(part 1 of 2)
# Autodesk Inventor assembly: 110033226_iam_11_農田
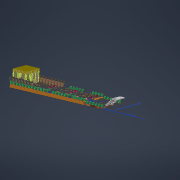
[picture p0: Inventor's stored thumbnail of the model, 180x180]
Saved by Autodesk Inventor 2022 (Build 260153000, 153)
## iProperties
Created: 2022-06-28
Part Number: 110033226_iam_11_農田
Document SubType Name: Assembly
Designer: User
Author: User
## Documents named in this file (13)
- D:\D-disk\pomelo\大一\下學期\機械設計製圖\1100332260_LEGOproj_沒有公主城堡\110033226_iam_11_農田.iam
- D:\D-disk\pomelo\大一\下學期\機械設計製圖\1100332260_LEGOproj_沒有公主城堡\110033226_ipt_44_農田基地.ipt
- D:\D-disk\pomelo\大一\下學期\機械設計製圖\1100332260_LEGOproj_沒有公主城堡\110033226_ipt_21_柵欄.ipt
- D:\D-disk\pomelo\大一\下學期\機械設計製圖\1100332260_LEGOproj_沒有公主城堡\110033226_ipt_04_小河.ipt
- D:\D-disk\pomelo\大一\下學期\機械設計製圖\1100332260_LEGOproj_沒有公主城堡\110033226_ipt_07_磚塊樺木(2x1).ipt
- D:\D-disk\pomelo\大一\下學期\機械設計製圖\1100332260_LEGOproj_沒有公主城堡\110033226_ipt_13_草地二.ipt
- D:\D-disk\pomelo\大一\下學期\機械設計製圖\1100332260_LEGOproj_沒有公主城堡\110033226_ipt_06_磚塊樺木(1x1).ipt
- D:\D-disk\pomelo\大一\下學期\機械設計製圖\1100332260_LEGOproj_沒有公主城堡\110033226_ipt_12_平滑面(2x1).ipt
- D:\D-disk\pomelo\大一\下學期\機械設計製圖\1100332260_LEGOproj_沒有公主城堡\110033226_ipt_08_平滑面(3x1).ipt
- D:\D-disk\pomelo\大一\下學期\機械設計製圖\1100332260_LEGOproj_沒有公主城堡\110033226_ipt_38_小樹木.ipt
- D:\D-disk\pomelo\大一\下學期\機械設計製圖\1100332260_LEGOproj_沒有公主城堡\110033226_ipt_45_小農田基地.ipt
- D:\D-disk\pomelo\大一\下學期\機械設計製圖\1100332260_LEGOproj_沒有公主城堡\110033226_ipt_11_樓梯支架.ipt
- D:\D-disk\pomelo\大一\下學期\機械設計製圖\1100332260_LEGOproj_沒有公主城堡\110033226_ipt_37_小河方塊.ipt
## Components (828 placed, 12 different names)
1. 110033226_ipt_38_小樹木:1 — 貼合:91, 貼合:92, 貼合:93, 貼合:96
2. 110033226_ipt_45_小農田基地:1 — 貼合:99, 貼合:100, 貼合:101, 貼合:102, 貼合:103, 貼合:104, 貼合:105, 貼合:106, 貼合:107, 貼合:108, 貼合:109, 貼合:110, 貼合:111, 貼合:112, 貼合:113, 貼合:130, 貼合:131, 貼合:135, 貼合:136, 貼合:137, 貼合:138, 貼合:139, 貼合:140, 貼合:141, 貼合:142, 貼合:146
3. 110033226_ipt_21_柵欄:50 — 貼合:108, 貼合:109, 貼合:110
4. 110033226_ipt_44_農田基地:1 — 貼合:1, 貼合:2, 貼合:3, 貼合:99, 貼合:100, 貼合:101
5. 110033226_ipt_44_農田基地:2
6. 110033226_ipt_44_農田基地:3 — 貼合:4, 貼合:5, 貼合:6, 貼合:7, 貼合:8, 貼合:9, 貼合:10, 貼合:11, 貼合:12, 貼合:13, 貼合:14, 貼合:15, 貼合:16, 貼合:17, 貼合:18, 貼合:19, 貼合:21, 貼合:22, 貼合:24, 貼合:25, 貼合:26, 貼合:27, 貼合:28, 貼合:29, 貼合:30, 貼合:31, 貼合:32, 貼合:33, 貼合:34, 貼合:35, 貼合:36, 貼合:37, 貼合:38, 貼合:39, 貼合:40, 貼合:41, 貼合:42, 貼合:43, 貼合:44, 貼合:45, 貼合:46, 貼合:47, 貼合:48, 貼合:49, 貼合:50, 貼合:88, 貼合:89, 貼合:90, 貼合:91, 貼合:92, 貼合:93, 貼合:94, 貼合:95, 貼合:97, 貼合:98
7. 110033226_ipt_04_小河:1 — 貼合:5, 貼合:6, 貼合:7
8. 110033226_ipt_04_小河:4
9. 110033226_ipt_04_小河:5
10. 110033226_ipt_04_小河:6
11. 110033226_ipt_04_小河:7
12. 110033226_ipt_04_小河:8
13. 110033226_ipt_04_小河:9
14. 110033226_ipt_04_小河:10
15. 110033226_ipt_04_小河:11
16. 110033226_ipt_04_小河:12
17. 110033226_ipt_04_小河:13
18. 110033226_ipt_04_小河:14
19. 110033226_ipt_04_小河:3 — 貼合:8, 貼合:9, 貼合:20
20. 110033226_ipt_04_小河:15 — 貼合:23
21. 110033226_ipt_04_小河:16
22. 110033226_ipt_04_小河:17
23. 110033226_ipt_04_小河:18
24. 110033226_ipt_04_小河:19
25. 110033226_ipt_04_小河:20
26. 110033226_ipt_04_小河:21
27. 110033226_ipt_04_小河:22
28. 110033226_ipt_04_小河:23
29. 110033226_ipt_04_小河:24
30. 110033226_ipt_04_小河:25
31. 110033226_ipt_21_柵欄:15 — 貼合:21, 貼合:22, 貼合:23
32. 110033226_ipt_21_柵欄:27
33. 110033226_ipt_07_磚塊樺木(2x1):1 — 貼合:24, 貼合:25, 貼合:26
34. 110033226_ipt_07_磚塊樺木(2x1):6
35. 110033226_ipt_07_磚塊樺木(2x1):7
36. 110033226_ipt_07_磚塊樺木(2x1):8
37. 110033226_ipt_07_磚塊樺木(2x1):9
38. 110033226_ipt_07_磚塊樺木(2x1):10
39. 110033226_ipt_07_磚塊樺木(2x1):11
40. 110033226_ipt_07_磚塊樺木(2x1):12
41. 110033226_ipt_07_磚塊樺木(2x1):13
42. 110033226_ipt_07_磚塊樺木(2x1):3 — 貼合:27, 貼合:28, 貼合:29
43. 110033226_ipt_07_磚塊樺木(2x1):14
44. 110033226_ipt_07_磚塊樺木(2x1):15
45. 110033226_ipt_07_磚塊樺木(2x1):16
46. 110033226_ipt_07_磚塊樺木(2x1):17
47. 110033226_ipt_07_磚塊樺木(2x1):18
48. 110033226_ipt_07_磚塊樺木(2x1):19
49. 110033226_ipt_07_磚塊樺木(2x1):20
50. 110033226_ipt_07_磚塊樺木(2x1):21
51. 110033226_ipt_07_磚塊樺木(2x1):5 — 貼合:30, 貼合:31, 貼合:32
52. 110033226_ipt_07_磚塊樺木(2x1):22
53. 110033226_ipt_07_磚塊樺木(2x1):23
54. 110033226_ipt_07_磚塊樺木(2x1):24
55. 110033226_ipt_07_磚塊樺木(2x1):25
56. 110033226_ipt_07_磚塊樺木(2x1):26
57. 110033226_ipt_07_磚塊樺木(2x1):27
58. 110033226_ipt_07_磚塊樺木(2x1):28
59. 110033226_ipt_07_磚塊樺木(2x1):2 — 貼合:33, 貼合:34, 貼合:35
60. 110033226_ipt_07_磚塊樺木(2x1):29
61. 110033226_ipt_07_磚塊樺木(2x1):30
62. 110033226_ipt_07_磚塊樺木(2x1):31
63. 110033226_ipt_07_磚塊樺木(2x1):32
64. 110033226_ipt_07_磚塊樺木(2x1):33
65. 110033226_ipt_07_磚塊樺木(2x1):4 — 貼合:36, 貼合:37, 貼合:38
66. 110033226_ipt_07_磚塊樺木(2x1):34
67. 110033226_ipt_07_磚塊樺木(2x1):35
68. 110033226_ipt_13_草地二:1 — 貼合:39, 貼合:40, 貼合:41
69. 110033226_ipt_13_草地二:2
70. 110033226_ipt_13_草地二:3
71. 110033226_ipt_13_草地二:4
72. 110033226_ipt_13_草地二:5
73. 110033226_ipt_13_草地二:6
74. 110033226_ipt_13_草地二:7
75. 110033226_ipt_13_草地二:8
76. 110033226_ipt_13_草地二:9
77. 110033226_ipt_13_草地二:10
78. 110033226_ipt_13_草地二:12 — 貼合:42, 貼合:43, 貼合:44
79. 110033226_ipt_13_草地二:13
80. 110033226_ipt_13_草地二:14
81. 110033226_ipt_13_草地二:15
82. 110033226_ipt_13_草地二:16
83. 110033226_ipt_13_草地二:17
84. 110033226_ipt_13_草地二:18
85. 110033226_ipt_13_草地二:19
86. 110033226_ipt_13_草地二:20
87. 110033226_ipt_13_草地二:21
88. 110033226_ipt_13_草地二:11 — 貼合:45, 貼合:46, 貼合:47
89. 110033226_ipt_13_草地二:22
90. 110033226_ipt_13_草地二:23
91. 110033226_ipt_13_草地二:24
92. 110033226_ipt_13_草地二:25
93. 110033226_ipt_13_草地二:26
94. 110033226_ipt_07_磚塊樺木(2x1):38 — 貼合:48, 貼合:49, 貼合:51, 貼合:52, 貼合:77
95. 110033226_ipt_06_磚塊樺木(1x1):3 — 貼合:50, 貼合:51, 貼合:52
96. 110033226_ipt_07_磚塊樺木(2x1):39
97. 110033226_ipt_06_磚塊樺木(1x1):4
98. 110033226_ipt_07_磚塊樺木(2x1):40
99. 110033226_ipt_06_磚塊樺木(1x1):5
100. 110033226_ipt_07_磚塊樺木(2x1):41
101. 110033226_ipt_06_磚塊樺木(1x1):6
102. 110033226_ipt_07_磚塊樺木(2x1):42
103. 110033226_ipt_06_磚塊樺木(1x1):7
104. 110033226_ipt_07_磚塊樺木(2x1):43
105. 110033226_ipt_06_磚塊樺木(1x1):8 — 貼合:62, 貼合:63, 貼合:64
106. 110033226_ipt_07_磚塊樺木(2x1):44
107. 110033226_ipt_06_磚塊樺木(1x1):9 — 貼合:60
108. 110033226_ipt_07_磚塊樺木(2x1):45
109. 110033226_ipt_06_磚塊樺木(1x1):10 — 貼合:59, 貼合:61
110. 110033226_ipt_07_磚塊樺木(2x1):46 — 貼合:55, 貼合:56
111. 110033226_ipt_06_磚塊樺木(1x1):11 — 貼合:53, 貼合:54
112. 110033226_ipt_07_磚塊樺木(2x1):47 — 貼合:78, 貼合:80, 貼合:81
113. 110033226_ipt_06_磚塊樺木(1x1):12
114. 110033226_ipt_07_磚塊樺木(2x1):48
115. 110033226_ipt_06_磚塊樺木(1x1):13
116. 110033226_ipt_07_磚塊樺木(2x1):49
117. 110033226_ipt_06_磚塊樺木(1x1):14
118. 110033226_ipt_07_磚塊樺木(2x1):50
119. 110033226_ipt_06_磚塊樺木(1x1):15
120. 110033226_ipt_07_磚塊樺木(2x1):51
121. 110033226_ipt_06_磚塊樺木(1x1):16
122. 110033226_ipt_07_磚塊樺木(2x1):52
123. 110033226_ipt_06_磚塊樺木(1x1):17
124. 110033226_ipt_07_磚塊樺木(2x1):53 — 貼合:86
125. 110033226_ipt_06_磚塊樺木(1x1):18
126. 110033226_ipt_07_磚塊樺木(2x1):54 — 貼合:85, 貼合:87
127. 110033226_ipt_06_磚塊樺木(1x1):19
128. 110033226_ipt_07_磚塊樺木(2x1):55
129. 110033226_ipt_06_磚塊樺木(1x1):20
130. 110033226_ipt_07_磚塊樺木(2x1):56 — 貼合:69, 貼合:71, 貼合:72, 貼合:73
131. 110033226_ipt_06_磚塊樺木(1x1):21
132. 110033226_ipt_07_磚塊樺木(2x1):57
133. 110033226_ipt_06_磚塊樺木(1x1):22
134. 110033226_ipt_07_磚塊樺木(2x1):58
135. 110033226_ipt_06_磚塊樺木(1x1):23
136. 110033226_ipt_07_磚塊樺木(2x1):59
137. 110033226_ipt_06_磚塊樺木(1x1):24
138. 110033226_ipt_07_磚塊樺木(2x1):60
139. 110033226_ipt_06_磚塊樺木(1x1):25
140. 110033226_ipt_07_磚塊樺木(2x1):61
141. 110033226_ipt_06_磚塊樺木(1x1):26 — 貼合:82
142. 110033226_ipt_07_磚塊樺木(2x1):62
143. 110033226_ipt_06_磚塊樺木(1x1):27
144. 110033226_ipt_07_磚塊樺木(2x1):63
145. 110033226_ipt_06_磚塊樺木(1x1):28
146. 110033226_ipt_07_磚塊樺木(2x1):64
147. 110033226_ipt_06_磚塊樺木(1x1):29
148. 110033226_ipt_07_磚塊樺木(2x1):65 — 貼合:68, 貼合:70
149. 110033226_ipt_06_磚塊樺木(1x1):30
150. 110033226_ipt_07_磚塊樺木(2x1):66
151. 110033226_ipt_06_磚塊樺木(1x1):31
152. 110033226_ipt_07_磚塊樺木(2x1):67
153. 110033226_ipt_06_磚塊樺木(1x1):32
154. 110033226_ipt_07_磚塊樺木(2x1):68
155. 110033226_ipt_06_磚塊樺木(1x1):33
156. 110033226_ipt_07_磚塊樺木(2x1):69
157. 110033226_ipt_06_磚塊樺木(1x1):34
158. 110033226_ipt_07_磚塊樺木(2x1):70
159. 110033226_ipt_06_磚塊樺木(1x1):35
160. 110033226_ipt_07_磚塊樺木(2x1):71
161. 110033226_ipt_06_磚塊樺木(1x1):36
162. 110033226_ipt_07_磚塊樺木(2x1):72
163. 110033226_ipt_06_磚塊樺木(1x1):37
164. 110033226_ipt_07_磚塊樺木(2x1):73
165. 110033226_ipt_06_磚塊樺木(1x1):38
166. 110033226_ipt_07_磚塊樺木(2x1):36 — 貼合:53, 貼合:54, 貼合:55, 貼合:57, 貼合:58
167. 110033226_ipt_06_磚塊樺木(1x1):1 — 貼合:56, 貼合:57, 貼合:58
168. 110033226_ipt_07_磚塊樺木(2x1):74
169. 110033226_ipt_06_磚塊樺木(1x1):39
170. 110033226_ipt_07_磚塊樺木(2x1):75
171. 110033226_ipt_06_磚塊樺木(1x1):40
172. 110033226_ipt_07_磚塊樺木(2x1):76
173. 110033226_ipt_06_磚塊樺木(1x1):41
174. 110033226_ipt_07_磚塊樺木(2x1):77
175. 110033226_ipt_06_磚塊樺木(1x1):42
176. 110033226_ipt_07_磚塊樺木(2x1):78
177. 110033226_ipt_06_磚塊樺木(1x1):43
178. 110033226_ipt_07_磚塊樺木(2x1):79
179. 110033226_ipt_06_磚塊樺木(1x1):44
180. 110033226_ipt_07_磚塊樺木(2x1):80
181. 110033226_ipt_06_磚塊樺木(1x1):45
182. 110033226_ipt_07_磚塊樺木(2x1):81
183. 110033226_ipt_06_磚塊樺木(1x1):46
184. 110033226_ipt_07_磚塊樺木(2x1):82
185. 110033226_ipt_06_磚塊樺木(1x1):47
186. 110033226_ipt_07_磚塊樺木(2x1):83
187. 110033226_ipt_06_磚塊樺木(1x1):48
188. 110033226_ipt_07_磚塊樺木(2x1):84 — 貼合:74, 貼合:75, 貼合:76
189. 110033226_ipt_06_磚塊樺木(1x1):49
190. 110033226_ipt_07_磚塊樺木(2x1):85
191. 110033226_ipt_06_磚塊樺木(1x1):50 — 貼合:83, 貼合:84
192. 110033226_ipt_07_磚塊樺木(2x1):86
193. 110033226_ipt_06_磚塊樺木(1x1):51
194. 110033226_ipt_07_磚塊樺木(2x1):87
195. 110033226_ipt_06_磚塊樺木(1x1):52
196. 110033226_ipt_07_磚塊樺木(2x1):88
197. 110033226_ipt_06_磚塊樺木(1x1):53
198. 110033226_ipt_07_磚塊樺木(2x1):89
199. 110033226_ipt_06_磚塊樺木(1x1):54
200. 110033226_ipt_07_磚塊樺木(2x1):90
201. 110033226_ipt_06_磚塊樺木(1x1):55
202. 110033226_ipt_07_磚塊樺木(2x1):91
203. 110033226_ipt_06_磚塊樺木(1x1):56
204. 110033226_ipt_07_磚塊樺木(2x1):92
205. 110033226_ipt_06_磚塊樺木(1x1):57
206. 110033226_ipt_07_磚塊樺木(2x1):93
207. 110033226_ipt_06_磚塊樺木(1x1):58
208. 110033226_ipt_07_磚塊樺木(2x1):94
209. 110033226_ipt_06_磚塊樺木(1x1):59
210. 110033226_ipt_07_磚塊樺木(2x1):95
211. 110033226_ipt_06_磚塊樺木(1x1):60
212. 110033226_ipt_07_磚塊樺木(2x1):96
213. 110033226_ipt_06_磚塊樺木(1x1):61
214. 110033226_ipt_07_磚塊樺木(2x1):97
215. 110033226_ipt_06_磚塊樺木(1x1):62
216. 110033226_ipt_07_磚塊樺木(2x1):98
217. 110033226_ipt_06_磚塊樺木(1x1):63
218. 110033226_ipt_07_磚塊樺木(2x1):99
219. 110033226_ipt_06_磚塊樺木(1x1):64
220. 110033226_ipt_07_磚塊樺木(2x1):100
221. 110033226_ipt_06_磚塊樺木(1x1):65
222. 110033226_ipt_07_磚塊樺木(2x1):101
223. 110033226_ipt_06_磚塊樺木(1x1):66
224. 110033226_ipt_07_磚塊樺木(2x1):102
225. 110033226_ipt_06_磚塊樺木(1x1):67
226. 110033226_ipt_07_磚塊樺木(2x1):103
227. 110033226_ipt_06_磚塊樺木(1x1):68
228. 110033226_ipt_07_磚塊樺木(2x1):104
229. 110033226_ipt_06_磚塊樺木(1x1):69
230. 110033226_ipt_07_磚塊樺木(2x1):105
231. 110033226_ipt_06_磚塊樺木(1x1):70
232. 110033226_ipt_07_磚塊樺木(2x1):106
233. 110033226_ipt_06_磚塊樺木(1x1):71
234. 110033226_ipt_07_磚塊樺木(2x1):107
235. 110033226_ipt_06_磚塊樺木(1x1):72
236. 110033226_ipt_07_磚塊樺木(2x1):108
237. 110033226_ipt_06_磚塊樺木(1x1):73
238. 110033226_ipt_07_磚塊樺木(2x1):109
239. 110033226_ipt_06_磚塊樺木(1x1):74
240. 110033226_ipt_07_磚塊樺木(2x1):110
241. 110033226_ipt_06_磚塊樺木(1x1):75
242. 110033226_ipt_07_磚塊樺木(2x1):111
243. 110033226_ipt_06_磚塊樺木(1x1):76
244. 110033226_ipt_07_磚塊樺木(2x1):112
245. 110033226_ipt_06_磚塊樺木(1x1):77
246. 110033226_ipt_07_磚塊樺木(2x1):113
247. 110033226_ipt_06_磚塊樺木(1x1):78
248. 110033226_ipt_07_磚塊樺木(2x1):114
249. 110033226_ipt_06_磚塊樺木(1x1):79
250. 110033226_ipt_07_磚塊樺木(2x1):115
251. 110033226_ipt_06_磚塊樺木(1x1):80
252. 110033226_ipt_07_磚塊樺木(2x1):116
253. 110033226_ipt_06_磚塊樺木(1x1):81
254. 110033226_ipt_07_磚塊樺木(2x1):117
255. 110033226_ipt_06_磚塊樺木(1x1):82
256. 110033226_ipt_07_磚塊樺木(2x1):118
257. 110033226_ipt_06_磚塊樺木(1x1):83
258. 110033226_ipt_07_磚塊樺木(2x1):119
259. 110033226_ipt_06_磚塊樺木(1x1):84
260. 110033226_ipt_07_磚塊樺木(2x1):120
261. 110033226_ipt_06_磚塊樺木(1x1):85
262. 110033226_ipt_07_磚塊樺木(2x1):184 — 貼合:68, 貼合:69, 貼合:70
263. 110033226_ipt_06_磚塊樺木(1x1):133 — 貼合:71, 貼合:72, 貼合:73
264. 110033226_ipt_07_磚塊樺木(2x1):185
265. 110033226_ipt_06_磚塊樺木(1x1):134
266. 110033226_ipt_07_磚塊樺木(2x1):186
267. 110033226_ipt_06_磚塊樺木(1x1):135
268. 110033226_ipt_07_磚塊樺木(2x1):187
269. 110033226_ipt_06_磚塊樺木(1x1):136
270. 110033226_ipt_07_磚塊樺木(2x1):188
271. 110033226_ipt_06_磚塊樺木(1x1):137
272. 110033226_ipt_07_磚塊樺木(2x1):189
273. 110033226_ipt_06_磚塊樺木(1x1):138
274. 110033226_ipt_07_磚塊樺木(2x1):190
275. 110033226_ipt_06_磚塊樺木(1x1):139
276. 110033226_ipt_07_磚塊樺木(2x1):191
277. 110033226_ipt_06_磚塊樺木(1x1):140
278. 110033226_ipt_07_磚塊樺木(2x1):192
279. 110033226_ipt_06_磚塊樺木(1x1):141
280. 110033226_ipt_07_磚塊樺木(2x1):193
281. 110033226_ipt_06_磚塊樺木(1x1):142
282. 110033226_ipt_07_磚塊樺木(2x1):194
283. 110033226_ipt_06_磚塊樺木(1x1):143
284. 110033226_ipt_07_磚塊樺木(2x1):195
285. 110033226_ipt_06_磚塊樺木(1x1):144
286. 110033226_ipt_07_磚塊樺木(2x1):196
287. 110033226_ipt_06_磚塊樺木(1x1):145
288. 110033226_ipt_07_磚塊樺木(2x1):197
289. 110033226_ipt_06_磚塊樺木(1x1):146
290. 110033226_ipt_07_磚塊樺木(2x1):198
291. 110033226_ipt_06_磚塊樺木(1x1):147
292. 110033226_ipt_07_磚塊樺木(2x1):199
293. 110033226_ipt_06_磚塊樺木(1x1):148
294. 110033226_ipt_07_磚塊樺木(2x1):200
295. 110033226_ipt_06_磚塊樺木(1x1):149
296. 110033226_ipt_07_磚塊樺木(2x1):201
297. 110033226_ipt_06_磚塊樺木(1x1):150
298. 110033226_ipt_07_磚塊樺木(2x1):202
299. 110033226_ipt_06_磚塊樺木(1x1):151
300. 110033226_ipt_07_磚塊樺木(2x1):203
301. 110033226_ipt_06_磚塊樺木(1x1):152
302. 110033226_ipt_07_磚塊樺木(2x1):204
303. 110033226_ipt_06_磚塊樺木(1x1):153
304. 110033226_ipt_07_磚塊樺木(2x1):205
305. 110033226_ipt_06_磚塊樺木(1x1):154
306. 110033226_ipt_07_磚塊樺木(2x1):206
307. 110033226_ipt_06_磚塊樺木(1x1):155
308. 110033226_ipt_07_磚塊樺木(2x1):207
309. 110033226_ipt_06_磚塊樺木(1x1):156
310. 110033226_ipt_08_平滑面(3x1):1 — 貼合:77, 貼合:78, 貼合:79
311. 110033226_ipt_08_平滑面(3x1):2
312. 110033226_ipt_08_平滑面(3x1):3
313. 110033226_ipt_08_平滑面(3x1):4
314. 110033226_ipt_08_平滑面(3x1):5
315. 110033226_ipt_08_平滑面(3x1):6
316. 110033226_ipt_08_平滑面(3x1):7
317. 110033226_ipt_08_平滑面(3x1):8
318. 110033226_ipt_08_平滑面(3x1):9 — 貼合:80, 貼合:81
319. 110033226_ipt_08_平滑面(3x1):10
320. 110033226_ipt_08_平滑面(3x1):11 — 貼合:82, 貼合:83, 貼合:84
321. 110033226_ipt_08_平滑面(3x1):12
322. 110033226_ipt_08_平滑面(3x1):13
323. 110033226_ipt_08_平滑面(3x1):14
324. 110033226_ipt_08_平滑面(3x1):15
325. 110033226_ipt_08_平滑面(3x1):16
326. 110033226_ipt_08_平滑面(3x1):17
327. 110033226_ipt_08_平滑面(3x1):18
328. 110033226_ipt_08_平滑面(3x1):19
329. 110033226_ipt_08_平滑面(3x1):20
330. 110033226_ipt_08_平滑面(3x1):21
331. 110033226_ipt_08_平滑面(3x1):22
332. 110033226_ipt_08_平滑面(3x1):23
333. 110033226_ipt_08_平滑面(3x1):24
334. 110033226_ipt_07_磚塊樺木(2x1):208 — 貼合:85, 貼合:86, 貼合:87
335. 110033226_ipt_07_磚塊樺木(2x1):209
336. 110033226_ipt_07_磚塊樺木(2x1):210
337. 110033226_ipt_07_磚塊樺木(2x1):211
338. 110033226_ipt_07_磚塊樺木(2x1):212
339. 110033226_ipt_07_磚塊樺木(2x1):213
340. 110033226_ipt_07_磚塊樺木(2x1):214
341. 110033226_ipt_07_磚塊樺木(2x1):215
342. 110033226_ipt_07_磚塊樺木(2x1):216
343. 110033226_ipt_07_磚塊樺木(2x1):217
344. 110033226_ipt_07_磚塊樺木(2x1):218
345. 110033226_ipt_07_磚塊樺木(2x1):219
346. 110033226_ipt_38_小樹木:2 — 貼合:88, 貼合:89, 貼合:90
347. 110033226_ipt_38_小樹木:3 — 對稱:1
348. 110033226_ipt_38_小樹木:5 — 貼合:94, 貼合:95, 貼合:96
349. 110033226_ipt_38_小樹木:6
350. 110033226_ipt_38_小樹木:7
351. 110033226_ipt_38_小樹木:8
352. 110033226_ipt_38_小樹木:9
353. 110033226_ipt_38_小樹木:10
354. 110033226_ipt_38_小樹木:11
355. 110033226_ipt_38_小樹木:4 — 貼合:97, 對稱:1, 貼合:98
356. 110033226_ipt_38_小樹木:12
357. 110033226_ipt_38_小樹木:13
358. 110033226_ipt_38_小樹木:14
359. 110033226_ipt_38_小樹木:15
360. 110033226_ipt_38_小樹木:16
361. 110033226_ipt_38_小樹木:17
362. 110033226_ipt_38_小樹木:18
363. 110033226_ipt_38_小樹木:19
364. 110033226_ipt_38_小樹木:20
365. 110033226_ipt_38_小樹木:21
366. 110033226_ipt_38_小樹木:22
367. 110033226_ipt_04_小河:26 — 貼合:102, 貼合:103, 貼合:104
368. 110033226_ipt_04_小河:27
369. 110033226_ipt_04_小河:28
370. 110033226_ipt_21_柵欄:49 — 貼合:105, 貼合:106, 貼合:107
371. 110033226_ipt_21_柵欄:51
372. 110033226_ipt_21_柵欄:52
373. 110033226_ipt_21_柵欄:53
374. 110033226_ipt_21_柵欄:54
375. 110033226_ipt_21_柵欄:55
376. 110033226_ipt_21_柵欄:56
377. 110033226_ipt_21_柵欄:57
378. 110033226_ipt_21_柵欄:58
379. 110033226_ipt_21_柵欄:59
380. 110033226_ipt_21_柵欄:60
381. 110033226_ipt_21_柵欄:61
382. 110033226_ipt_11_樓梯支架:1 — 貼合:111, 貼合:112, 貼合:113
383. 110033226_ipt_11_樓梯支架:4
384. 110033226_ipt_11_樓梯支架:5 — 貼合:119, 貼合:127
385. 110033226_ipt_11_樓梯支架:6 — 貼合:120, 貼合:126
386. 110033226_ipt_11_樓梯支架:7
387. 110033226_ipt_11_樓梯支架:8 — 貼合:117, 貼合:129
388. 110033226_ipt_11_樓梯支架:9 — 貼合:118, 貼合:128
389. 110033226_ipt_11_樓梯支架:10
390. 110033226_ipt_11_樓梯支架:11
391. 110033226_ipt_11_樓梯支架:12 — 貼合:114, 貼合:115, 貼合:116, 貼合:121, 貼合:125
392. 110033226_ipt_08_平滑面(3x1):25 — 貼合:114, 貼合:115, 貼合:116
393. 110033226_ipt_08_平滑面(3x1):26 — 貼合:122, 貼合:123, 貼合:124
394. 110033226_ipt_08_平滑面(3x1):27 — 貼合:122, 貼合:123, 貼合:124
395. 110033226_ipt_08_平滑面(3x1):33
396. 110033226_ipt_08_平滑面(3x1):34
397. 110033226_ipt_08_平滑面(3x1):35
398. 110033226_ipt_08_平滑面(3x1):29 — 貼合:121, 貼合:125
399. 110033226_ipt_08_平滑面(3x1):36
400. 110033226_ipt_08_平滑面(3x1):28 — 貼合:120, 貼合:126
401. 110033226_ipt_08_平滑面(3x1):37
402. 110033226_ipt_08_平滑面(3x1):31 — 貼合:119, 貼合:127
403. 110033226_ipt_08_平滑面(3x1):38
404. 110033226_ipt_08_平滑面(3x1):30 — 貼合:118, 貼合:128
405. 110033226_ipt_08_平滑面(3x1):39
406. 110033226_ipt_08_平滑面(3x1):32 — 貼合:117, 貼合:129
407. 110033226_ipt_08_平滑面(3x1):40
408. 110033226_ipt_04_小河:29 — 貼合:130, 貼合:131
409. 110033226_ipt_04_小河:30
410. 110033226_ipt_04_小河:31
411. 110033226_ipt_04_小河:32 — 貼合:144, 貼合:145
412. 110033226_ipt_04_小河:33
413. 110033226_ipt_04_小河:34
414. 110033226_ipt_04_小河:35
415. 110033226_ipt_04_小河:36
416. 110033226_ipt_04_小河:37
417. 110033226_ipt_04_小河:38
418. 110033226_ipt_04_小河:39
419. 110033226_ipt_04_小河:40
420. 110033226_ipt_04_小河:41
421. 110033226_ipt_04_小河:42
422. 110033226_ipt_04_小河:43
423. 110033226_ipt_04_小河:44
424. 110033226_ipt_04_小河:45
425. 110033226_ipt_04_小河:46
426. 110033226_ipt_04_小河:47 — 貼合:132, 貼合:133, 貼合:134
427. 110033226_ipt_04_小河:48
428. 110033226_ipt_04_小河:49
429. 110033226_ipt_04_小河:50
430. 110033226_ipt_04_小河:51
431. 110033226_ipt_04_小河:52
432. 110033226_ipt_04_小河:53
433. 110033226_ipt_04_小河:54
434. 110033226_ipt_04_小河:55
435. 110033226_ipt_04_小河:56 — 貼合:132, 貼合:133, 貼合:134
436. 110033226_ipt_04_小河:57
437. 110033226_ipt_04_小河:58
438. 110033226_ipt_04_小河:59
439. 110033226_ipt_04_小河:60
440. 110033226_ipt_04_小河:61
441. 110033226_ipt_04_小河:62
442. 110033226_ipt_04_小河:63 — 貼合:135, 貼合:136, 貼合:137
443. 110033226_ipt_04_小河:65
444. 110033226_ipt_04_小河:66
445. 110033226_ipt_04_小河:64 — 貼合:138, 貼合:139, 貼合:140
446. 110033226_ipt_04_小河:67 — 貼合:143
447. 110033226_ipt_37_小河方塊:1 — 貼合:141, 貼合:142, 貼合:143
448. 110033226_ipt_37_小河方塊:2
449. 110033226_ipt_37_小河方塊:3
450. 110033226_ipt_37_小河方塊:4
451. 110033226_ipt_37_小河方塊:5 — 貼合:144, 貼合:145, 貼合:146
452. 110033226_ipt_37_小河方塊:6
453. 110033226_ipt_37_小河方塊:7
454. 110033226_ipt_37_小河方塊:8
455. 110033226_ipt_21_柵欄:14 — 貼合:18, 貼合:19, 貼合:20
456. 110033226_ipt_21_柵欄:24
457. 110033226_ipt_21_柵欄:25
458. 110033226_ipt_21_柵欄:26
459. 110033226_ipt_21_柵欄:1 — 貼合:4, 貼合:10, 貼合:11
460. 110033226_ipt_21_柵欄:2
461. 110033226_ipt_21_柵欄:3
462. 110033226_ipt_21_柵欄:4
463. 110033226_ipt_21_柵欄:5
464. 110033226_ipt_21_柵欄:6
465. 110033226_ipt_21_柵欄:7
466. 110033226_ipt_21_柵欄:8
467. 110033226_ipt_21_柵欄:9
468. 110033226_ipt_21_柵欄:10
469. 110033226_ipt_21_柵欄:11
470. 110033226_ipt_21_柵欄:12
471. 110033226_ipt_21_柵欄:16 — 貼合:15, 貼合:16, 貼合:17
472. 110033226_ipt_21_柵欄:20
473. 110033226_ipt_21_柵欄:21
474. 110033226_ipt_21_柵欄:22
475. 110033226_ipt_21_柵欄:23
476. 110033226_ipt_21_柵欄:13 — 貼合:12, 貼合:13, 貼合:14
477. 110033226_ipt_21_柵欄:17
478. 110033226_ipt_21_柵欄:18
479. 110033226_ipt_21_柵欄:19
480. 110033226_ipt_21_柵欄:28
481. 110033226_ipt_21_柵欄:29
482. 110033226_ipt_21_柵欄:30
483. 110033226_ipt_21_柵欄:31
484. 110033226_ipt_21_柵欄:32
485. 110033226_ipt_21_柵欄:33
486. 110033226_ipt_21_柵欄:34
487. 110033226_ipt_21_柵欄:35
488. 110033226_ipt_21_柵欄:36
489. 110033226_ipt_21_柵欄:37
490. 110033226_ipt_21_柵欄:38
491. 110033226_ipt_21_柵欄:39
492. 110033226_ipt_21_柵欄:40
493. 110033226_ipt_21_柵欄:41
494. 110033226_ipt_21_柵欄:42
495. 110033226_ipt_21_柵欄:43
496. 110033226_ipt_21_柵欄:44
497. 110033226_ipt_21_柵欄:45
498. 110033226_ipt_21_柵欄:46
499. 110033226_ipt_21_柵欄:47
500. 110033226_ipt_21_柵欄:48
501. 110033226_ipt_07_磚塊樺木(2x1):37 — 貼合:59, 貼合:60, 貼合:61
502. 110033226_ipt_06_磚塊樺木(1x1):2 — 貼合:62, 貼合:63, 貼合:64
503. 110033226_ipt_07_磚塊樺木(2x1):121
504. 110033226_ipt_06_磚塊樺木(1x1):86
505. 110033226_ipt_07_磚塊樺木(2x1):122
506. 110033226_ipt_06_磚塊樺木(1x1):87
507. 110033226_ipt_07_磚塊樺木(2x1):123
508. 110033226_ipt_06_磚塊樺木(1x1):88
509. 110033226_ipt_07_磚塊樺木(2x1):124
510. 110033226_ipt_06_磚塊樺木(1x1):89
511. 110033226_ipt_07_磚塊樺木(2x1):125
512. 110033226_ipt_06_磚塊樺木(1x1):90
513. 110033226_ipt_07_磚塊樺木(2x1):126
514. 110033226_ipt_06_磚塊樺木(1x1):91
515. 110033226_ipt_07_磚塊樺木(2x1):127
516. 110033226_ipt_06_磚塊樺木(1x1):92
517. 110033226_ipt_07_磚塊樺木(2x1):128
518. 110033226_ipt_06_磚塊樺木(1x1):93
519. 110033226_ipt_07_磚塊樺木(2x1):129
520. 110033226_ipt_06_磚塊樺木(1x1):94
521. 110033226_ipt_07_磚塊樺木(2x1):130
522. 110033226_ipt_06_磚塊樺木(1x1):95
523. 110033226_ipt_07_磚塊樺木(2x1):131
524. 110033226_ipt_06_磚塊樺木(1x1):96 — 貼合:65, 貼合:66
525. 110033226_ipt_07_磚塊樺木(2x1):132
526. 110033226_ipt_06_磚塊樺木(1x1):97 — 貼合:79
527. 110033226_ipt_07_磚塊樺木(2x1):133
528. 110033226_ipt_06_磚塊樺木(1x1):98
529. 110033226_ipt_07_磚塊樺木(2x1):134
530. 110033226_ipt_06_磚塊樺木(1x1):99
531. 110033226_ipt_07_磚塊樺木(2x1):135
532. 110033226_ipt_06_磚塊樺木(1x1):100
533. 110033226_ipt_07_磚塊樺木(2x1):136
534. 110033226_ipt_06_磚塊樺木(1x1):101
535. 110033226_ipt_07_磚塊樺木(2x1):137
536. 110033226_ipt_06_磚塊樺木(1x1):102
537. 110033226_ipt_07_磚塊樺木(2x1):138
538. 110033226_ipt_06_磚塊樺木(1x1):103
539. 110033226_ipt_07_磚塊樺木(2x1):139
540. 110033226_ipt_06_磚塊樺木(1x1):104
541. 110033226_ipt_07_磚塊樺木(2x1):140
542. 110033226_ipt_06_磚塊樺木(1x1):105
543. 110033226_ipt_07_磚塊樺木(2x1):141
544. 110033226_ipt_06_磚塊樺木(1x1):106
545. 110033226_ipt_07_磚塊樺木(2x1):142
546. 110033226_ipt_06_磚塊樺木(1x1):107
547. 110033226_ipt_07_磚塊樺木(2x1):143 — 貼合:67
548. 110033226_ipt_06_磚塊樺木(1x1):108
549. 110033226_ipt_07_磚塊樺木(2x1):152
550. 110033226_ipt_06_磚塊樺木(1x1):109
551. 110033226_ipt_07_磚塊樺木(2x1):153
552. 110033226_ipt_06_磚塊樺木(1x1):110
553. 110033226_ipt_07_磚塊樺木(2x1):154
554. 110033226_ipt_06_磚塊樺木(1x1):111
555. 110033226_ipt_07_磚塊樺木(2x1):155
556. 110033226_ipt_06_磚塊樺木(1x1):112
557. 110033226_ipt_07_磚塊樺木(2x1):156
558. 110033226_ipt_06_磚塊樺木(1x1):113
559. 110033226_ipt_07_磚塊樺木(2x1):157
560. 110033226_ipt_06_磚塊樺木(1x1):114
561. 110033226_ipt_07_磚塊樺木(2x1):158
562. 110033226_ipt_06_磚塊樺木(1x1):115
563. 110033226_ipt_07_磚塊樺木(2x1):159
564. 110033226_ipt_06_磚塊樺木(1x1):116
565. 110033226_ipt_07_磚塊樺木(2x1):160
566. 110033226_ipt_06_磚塊樺木(1x1):117
567. 110033226_ipt_07_磚塊樺木(2x1):161
568. 110033226_ipt_06_磚塊樺木(1x1):118
569. 110033226_ipt_07_磚塊樺木(2x1):162
570. 110033226_ipt_06_磚塊樺木(1x1):119
571. 110033226_ipt_07_磚塊樺木(2x1):163
572. 110033226_ipt_06_磚塊樺木(1x1):120
573. 110033226_ipt_07_磚塊樺木(2x1):164
574. 110033226_ipt_06_磚塊樺木(1x1):121
575. 110033226_ipt_07_磚塊樺木(2x1):165
576. 110033226_ipt_06_磚塊樺木(1x1):122
577. 110033226_ipt_07_磚塊樺木(2x1):166
578. 110033226_ipt_06_磚塊樺木(1x1):123
579. 110033226_ipt_07_磚塊樺木(2x1):167
580. 110033226_ipt_06_磚塊樺木(1x1):124
581. 110033226_ipt_07_磚塊樺木(2x1):168
582. 110033226_ipt_06_磚塊樺木(1x1):125
583. 110033226_ipt_07_磚塊樺木(2x1):169
584. 110033226_ipt_06_磚塊樺木(1x1):126
585. 110033226_ipt_07_磚塊樺木(2x1):170
586. 110033226_ipt_06_磚塊樺木(1x1):127
587. 110033226_ipt_07_磚塊樺木(2x1):171
588. 110033226_ipt_06_磚塊樺木(1x1):128
589. 110033226_ipt_07_磚塊樺木(2x1):172
590. 110033226_ipt_06_磚塊樺木(1x1):129
591. 110033226_ipt_07_磚塊樺木(2x1):173
592. 110033226_ipt_06_磚塊樺木(1x1):130
593. 110033226_ipt_07_磚塊樺木(2x1):174
594. 110033226_ipt_06_磚塊樺木(1x1):131
595. 110033226_ipt_07_磚塊樺木(2x1):175
596. 110033226_ipt_06_磚塊樺木(1x1):132
597. 110033226_ipt_12_平滑面(2x1):1 — 貼合:74, 貼合:75, 貼合:76
598. 110033226_ipt_12_平滑面(2x1):3
599. 110033226_ipt_12_平滑面(2x1):4
600. 110033226_ipt_12_平滑面(2x1):5
601. 110033226_ipt_12_平滑面(2x1):6
602. 110033226_ipt_12_平滑面(2x1):7
603. 110033226_ipt_12_平滑面(2x1):8
604. 110033226_ipt_12_平滑面(2x1):9
605. 110033226_ipt_12_平滑面(2x1):10
606. 110033226_ipt_12_平滑面(2x1):11
607. 110033226_ipt_12_平滑面(2x1):12
608. 110033226_ipt_12_平滑面(2x1):13
609. 110033226_ipt_12_平滑面(2x1):14
610. 110033226_ipt_12_平滑面(2x1):15
611. 110033226_ipt_12_平滑面(2x1):16
612. 110033226_ipt_12_平滑面(2x1):17
613. 110033226_ipt_12_平滑面(2x1):18
614. 110033226_ipt_12_平滑面(2x1):19
615. 110033226_ipt_12_平滑面(2x1):20
616. 110033226_ipt_12_平滑面(2x1):21
617. 110033226_ipt_12_平滑面(2x1):22
618. 110033226_ipt_12_平滑面(2x1):23
619. 110033226_ipt_12_平滑面(2x1):24
620. 110033226_ipt_12_平滑面(2x1):25
621. 110033226_ipt_12_平滑面(2x1):26
622. 110033226_ipt_12_平滑面(2x1):27
623. 110033226_ipt_12_平滑面(2x1):28
624. 110033226_ipt_12_平滑面(2x1):29
625. 110033226_ipt_12_平滑面(2x1):30
626. 110033226_ipt_12_平滑面(2x1):31
627. 110033226_ipt_12_平滑面(2x1):32
628. 110033226_ipt_12_平滑面(2x1):33
629. 110033226_ipt_12_平滑面(2x1):34
630. 110033226_ipt_12_平滑面(2x1):35
631. 110033226_ipt_12_平滑面(2x1):36
632. 110033226_ipt_12_平滑面(2x1):37
633. 110033226_ipt_12_平滑面(2x1):38
634. 110033226_ipt_12_平滑面(2x1):39
635. 110033226_ipt_12_平滑面(2x1):40
636. 110033226_ipt_12_平滑面(2x1):41
637. 110033226_ipt_12_平滑面(2x1):42
638. 110033226_ipt_12_平滑面(2x1):43
639. 110033226_ipt_12_平滑面(2x1):44
640. 110033226_ipt_12_平滑面(2x1):45
641. 110033226_ipt_12_平滑面(2x1):46
642. 110033226_ipt_12_平滑面(2x1):47
643. 110033226_ipt_12_平滑面(2x1):48
644. 110033226_ipt_12_平滑面(2x1):49
645. 110033226_ipt_12_平滑面(2x1):50
646. 110033226_ipt_12_平滑面(2x1):51
647. 110033226_ipt_12_平滑面(2x1):52
648. 110033226_ipt_12_平滑面(2x1):53
649. 110033226_ipt_12_平滑面(2x1):54
650. 110033226_ipt_12_平滑面(2x1):55
651. 110033226_ipt_12_平滑面(2x1):56
652. 110033226_ipt_12_平滑面(2x1):57
653. 110033226_ipt_12_平滑面(2x1):58
654. 110033226_ipt_12_平滑面(2x1):59
655. 110033226_ipt_12_平滑面(2x1):60
656. 110033226_ipt_12_平滑面(2x1):61
657. 110033226_ipt_12_平滑面(2x1):62
658. 110033226_ipt_12_平滑面(2x1):63
659. 110033226_ipt_12_平滑面(2x1):64
660. 110033226_ipt_12_平滑面(2x1):65
661. 110033226_ipt_12_平滑面(2x1):66
662. 110033226_ipt_12_平滑面(2x1):67
663. 110033226_ipt_12_平滑面(2x1):68
664. 110033226_ipt_12_平滑面(2x1):69
665. 110033226_ipt_12_平滑面(2x1):70
666. 110033226_ipt_12_平滑面(2x1):71
667. 110033226_ipt_12_平滑面(2x1):72
668. 110033226_ipt_12_平滑面(2x1):73
669. 110033226_ipt_12_平滑面(2x1):74
670. 110033226_ipt_12_平滑面(2x1):75
671. 110033226_ipt_12_平滑面(2x1):76
672. 110033226_ipt_12_平滑面(2x1):77
673. 110033226_ipt_12_平滑面(2x1):78
674. 110033226_ipt_12_平滑面(2x1):79
675. 110033226_ipt_12_平滑面(2x1):80
676. 110033226_ipt_12_平滑面(2x1):81
677. 110033226_ipt_12_平滑面(2x1):82
678. 110033226_ipt_12_平滑面(2x1):83
679. 110033226_ipt_12_平滑面(2x1):84
680. 110033226_ipt_12_平滑面(2x1):85
681. 110033226_ipt_12_平滑面(2x1):86
682. 110033226_ipt_12_平滑面(2x1):87
683. 110033226_ipt_12_平滑面(2x1):88
684. 110033226_ipt_12_平滑面(2x1):89
685. 110033226_ipt_12_平滑面(2x1):90
686. 110033226_ipt_12_平滑面(2x1):91
687. 110033226_ipt_12_平滑面(2x1):92
688. 110033226_ipt_12_平滑面(2x1):93
689. 110033226_ipt_12_平滑面(2x1):94
690. 110033226_ipt_12_平滑面(2x1):95
691. 110033226_ipt_12_平滑面(2x1):96
692. 110033226_ipt_12_平滑面(2x1):97
693. 110033226_ipt_12_平滑面(2x1):98
694. 110033226_ipt_12_平滑面(2x1):99
695. 110033226_ipt_12_平滑面(2x1):100
696. 110033226_ipt_12_平滑面(2x1):101
697. 110033226_ipt_12_平滑面(2x1):102
698. 110033226_ipt_12_平滑面(2x1):103
699. 110033226_ipt_12_平滑面(2x1):104
700. 110033226_ipt_12_平滑面(2x1):105
701. 110033226_ipt_12_平滑面(2x1):106
702. 110033226_ipt_12_平滑面(2x1):107
703. 110033226_ipt_12_平滑面(2x1):108
704. 110033226_ipt_12_平滑面(2x1):109
705. 110033226_ipt_12_平滑面(2x1):110
706. 110033226_ipt_12_平滑面(2x1):111
707. 110033226_ipt_12_平滑面(2x1):112
708. 110033226_ipt_12_平滑面(2x1):113
709. 110033226_ipt_12_平滑面(2x1):114
710. 110033226_ipt_12_平滑面(2x1):115
711. 110033226_ipt_12_平滑面(2x1):116
712. 110033226_ipt_12_平滑面(2x1):117
713. 110033226_ipt_12_平滑面(2x1):118
714. 110033226_ipt_12_平滑面(2x1):119
715. 110033226_ipt_12_平滑面(2x1):120
716. 110033226_ipt_12_平滑面(2x1):121
717. 110033226_ipt_12_平滑面(2x1):122
718. 110033226_ipt_12_平滑面(2x1):123
719. 110033226_ipt_12_平滑面(2x1):124
720. 110033226_ipt_12_平滑面(2x1):125
721. 110033226_ipt_12_平滑面(2x1):126
722. 110033226_ipt_12_平滑面(2x1):127
723. 110033226_ipt_12_平滑面(2x1):128
724. 110033226_ipt_12_平滑面(2x1):129
725. 110033226_ipt_12_平滑面(2x1):130
726. 110033226_ipt_12_平滑面(2x1):131
727. 110033226_ipt_12_平滑面(2x1):132
728. 110033226_ipt_12_平滑面(2x1):133
729. 110033226_ipt_12_平滑面(2x1):134
730. 110033226_ipt_12_平滑面(2x1):135
731. 110033226_ipt_12_平滑面(2x1):136
732. 110033226_ipt_12_平滑面(2x1):137
733. 110033226_ipt_12_平滑面(2x1):138
734. 110033226_ipt_12_平滑面(2x1):139
735. 110033226_ipt_12_平滑面(2x1):140
736. 110033226_ipt_12_平滑面(2x1):141
737. 110033226_ipt_12_平滑面(2x1):142
738. 110033226_ipt_12_平滑面(2x1):143
739. 110033226_ipt_12_平滑面(2x1):144
740. 110033226_ipt_12_平滑面(2x1):145
741. 110033226_ipt_12_平滑面(2x1):146
742. 110033226_ipt_12_平滑面(2x1):147
743. 110033226_ipt_12_平滑面(2x1):148
744. 110033226_ipt_12_平滑面(2x1):149
745. 110033226_ipt_12_平滑面(2x1):150
746. 110033226_ipt_12_平滑面(2x1):151
747. 110033226_ipt_12_平滑面(2x1):152
748. 110033226_ipt_12_平滑面(2x1):153
749. 110033226_ipt_12_平滑面(2x1):154
750. 110033226_ipt_12_平滑面(2x1):155
751. 110033226_ipt_12_平滑面(2x1):156
752. 110033226_ipt_12_平滑面(2x1):157
753. 110033226_ipt_12_平滑面(2x1):158
754. 110033226_ipt_12_平滑面(2x1):159
755. 110033226_ipt_12_平滑面(2x1):160
756. 110033226_ipt_12_平滑面(2x1):161
757. 110033226_ipt_12_平滑面(2x1):162
758. 110033226_ipt_12_平滑面(2x1):163
759. 110033226_ipt_12_平滑面(2x1):164
760. 110033226_ipt_12_平滑面(2x1):165
761. 110033226_ipt_12_平滑面(2x1):166
762. 110033226_ipt_12_平滑面(2x1):167
763. 110033226_ipt_12_平滑面(2x1):168
764. 110033226_ipt_12_平滑面(2x1):169
765. 110033226_ipt_12_平滑面(2x1):170
766. 110033226_ipt_12_平滑面(2x1):171
767. 110033226_ipt_12_平滑面(2x1):172
768. 110033226_ipt_12_平滑面(2x1):173
769. 110033226_ipt_12_平滑面(2x1):174
770. 110033226_ipt_12_平滑面(2x1):175
771. 110033226_ipt_12_平滑面(2x1):176
772. 110033226_ipt_12_平滑面(2x1):177
773. 110033226_ipt_12_平滑面(2x1):178
774. 110033226_ipt_12_平滑面(2x1):179
775. 110033226_ipt_12_平滑面(2x1):180
776. 110033226_ipt_12_平滑面(2x1):181
777. 110033226_ipt_12_平滑面(2x1):182
778. 110033226_ipt_12_平滑面(2x1):183
779. 110033226_ipt_12_平滑面(2x1):184
780. 110033226_ipt_12_平滑面(2x1):185
781. 110033226_ipt_12_平滑面(2x1):186
782. 110033226_ipt_12_平滑面(2x1):187
783. 110033226_ipt_12_平滑面(2x1):188
784. 110033226_ipt_12_平滑面(2x1):189
785. 110033226_ipt_12_平滑面(2x1):190
786. 110033226_ipt_12_平滑面(2x1):191
787. 110033226_ipt_12_平滑面(2x1):192
788. 110033226_ipt_12_平滑面(2x1):193
789. 110033226_ipt_12_平滑面(2x1):194
790. 110033226_ipt_12_平滑面(2x1):195
791. 110033226_ipt_12_平滑面(2x1):196
792. 110033226_ipt_12_平滑面(2x1):197
793. 110033226_ipt_12_平滑面(2x1):198
794. 110033226_ipt_12_平滑面(2x1):199
795. 110033226_ipt_12_平滑面(2x1):200
796. 110033226_ipt_12_平滑面(2x1):201
797. 110033226_ipt_12_平滑面(2x1):202
798. 110033226_ipt_12_平滑面(2x1):203
799. 110033226_ipt_12_平滑面(2x1):204
800. 110033226_ipt_12_平滑面(2x1):205
801. 110033226_ipt_12_平滑面(2x1):206
802. 110033226_ipt_12_平滑面(2x1):207
803. 110033226_ipt_12_平滑面(2x1):208
804. 110033226_ipt_12_平滑面(2x1):209
805. 110033226_ipt_12_平滑面(2x1):210
806. 110033226_ipt_12_平滑面(2x1):211
807. 110033226_ipt_12_平滑面(2x1):212
808. 110033226_ipt_12_平滑面(2x1):213
809. 110033226_ipt_12_平滑面(2x1):214
810. 110033226_ipt_12_平滑面(2x1):215
811. 110033226_ipt_12_平滑面(2x1):216
812. 110033226_ipt_12_平滑面(2x1):217
813. 110033226_ipt_07_磚塊樺木(2x1):144 — 貼合:65, 貼合:66, 貼合:67
814. 110033226_ipt_07_磚塊樺木(2x1):145
815. 110033226_ipt_07_磚塊樺木(2x1):146
816. 110033226_ipt_07_磚塊樺木(2x1):147
817. 110033226_ipt_07_磚塊樺木(2x1):148
818. 110033226_ipt_07_磚塊樺木(2x1):149
819. 110033226_ipt_07_磚塊樺木(2x1):150
820. 110033226_ipt_07_磚塊樺木(2x1):151
821. 110033226_ipt_07_磚塊樺木(2x1):176
822. 110033226_ipt_07_磚塊樺木(2x1):177
823. 110033226_ipt_07_磚塊樺木(2x1):178
824. 110033226_ipt_07_磚塊樺木(2x1):179
825. 110033226_ipt_07_磚塊樺木(2x1):180
826. 110033226_ipt_07_磚塊樺木(2x1):181
827. 110033226_ipt_07_磚塊樺木(2x1):182
828. 110033226_ipt_07_磚塊樺木(2x1):183
## Component patterns: (3 elements, first: 110033226_ipt_44_農田基地:1), (12 elements, first: 110033226_ipt_04_小河:1), (12 elements, first: 110033226_ipt_04_小河:3), (2 elements), (2 elements, first: 110033226_ipt_21_柵欄:15), (2 elements), (9 elements, first: 110033226_ipt_07_磚塊樺木(2x1):1), (9 elements, first: 110033226_ipt_07_磚塊樺木(2x1):3), (8 elements, first: 110033226_ipt_07_磚塊樺木(2x1):5), (6 elements, first: 110033226_ipt_07_磚塊樺木(2x1):2), (3 elements, first: 110033226_ipt_07_磚塊樺木(2x1):4), (10 elements, first: 110033226_ipt_13_草地二:1), (10 elements, first: 110033226_ipt_13_草地二:12), (6 elements, first: 110033226_ipt_13_草地二:11), (36 elements, first: 110033226_ipt_07_磚塊樺木(2x1):38 + 110033226_ipt_06_磚塊樺木(1x1):3), (48 elements, first: 110033226_ipt_07_磚塊樺木(2x1):36 + 110033226_ipt_06_磚塊樺木(1x1):1), (2 elements), (24 elements, first: 110033226_ipt_07_磚塊樺木(2x1):184 + 110033226_ipt_06_磚塊樺木(1x1):133), (4 elements), (8 elements, first: 110033226_ipt_08_平滑面(3x1):1), (2 elements, first: 110033226_ipt_08_平滑面(3x1):9), (14 elements, first: 110033226_ipt_08_平滑面(3x1):11), (12 elements, first: 110033226_ipt_07_磚塊樺木(2x1):208), (2 elements, first: 110033226_ipt_38_小樹木:2), (7 elements, first: 110033226_ipt_38_小樹木:5), (12 elements, first: 110033226_ipt_38_小樹木:4), (3 elements, first: 110033226_ipt_04_小河:26), (12 elements, first: 110033226_ipt_21_柵欄:49), (10 elements, first: 110033226_ipt_11_樓梯支架:1), (2 elements, first: 110033226_ipt_08_平滑面(3x1):25), (4 elements, first: 110033226_ipt_08_平滑面(3x1):27), (2 elements, first: 110033226_ipt_08_平滑面(3x1):29), (2 elements, first: 110033226_ipt_08_平滑面(3x1):28), (2 elements, first: 110033226_ipt_08_平滑面(3x1):31), (2 elements, first: 110033226_ipt_08_平滑面(3x1):30), (2 elements, first: 110033226_ipt_08_平滑面(3x1):32), (27 elements, first: 110033226_ipt_04_小河:29), (7 elements, first: 110033226_ipt_04_小河:56), (3 elements, first: 110033226_ipt_04_小河:63), (2 elements, first: 110033226_ipt_04_小河:64), (4 elements, first: 110033226_ipt_37_小河方塊:1), (4 elements, first: 110033226_ipt_37_小河方塊:5), (2 elements, first: 110033226_ipt_21_柵欄:14), 元件陣列 7:2 (2 elements), (12 elements, first: 110033226_ipt_21_柵欄:1), (5 elements, first: 110033226_ipt_21_柵欄:16), (4 elements, first: 110033226_ipt_21_柵欄:13), 元件陣列 4:2 (12 elements), 元件陣列 6:2 (5 elements), 元件陣列 5:2 (4 elements), (24 elements, first: 110033226_ipt_07_磚塊樺木(2x1):37 + 110033226_ipt_06_磚塊樺木(1x1):2), (2 elements), 元件陣列 22:2 (24 elements), (2 elements), (54 elements, first: 110033226_ipt_12_平滑面(2x1):1), 元件陣列 27:2 (54 elements), 元件陣列 27:3 (54 elements), 元件陣列 27:4 (54 elements), (4 elements, first: 110033226_ipt_07_磚塊樺木(2x1):144), 元件陣列 23:2 (4 elements), 元件陣列 23:3 (4 elements), 元件陣列 23:4 (4 elements)
## Relationships (147: Mate 146, Symmetry 1)
- 貼合:1 [Mate]: 110033226_ipt_44_農田基地:1
- 貼合:2 [Mate]: 110033226_ipt_44_農田基地:1
- 貼合:3 [Mate]: 110033226_ipt_44_農田基地:1
- 貼合:4 [Mate]: 110033226_ipt_44_農田基地:3 ↔ 110033226_ipt_21_柵欄:1
- 貼合:5 [Mate]: 110033226_ipt_44_農田基地:3 ↔ 110033226_ipt_04_小河:1
- 貼合:6 [Mate]: 110033226_ipt_44_農田基地:3 ↔ 110033226_ipt_04_小河:1
- 貼合:7 [Mate]: 110033226_ipt_44_農田基地:3 ↔ 110033226_ipt_04_小河:1
- 貼合:8 [Mate]: 110033226_ipt_44_農田基地:3 ↔ 110033226_ipt_04_小河:3
- 貼合:9 [Mate]: 110033226_ipt_44_農田基地:3 ↔ 110033226_ipt_04_小河:3
- 貼合:10 [Mate]: 110033226_ipt_44_農田基地:3 ↔ 110033226_ipt_21_柵欄:1
- 貼合:11 [Mate]: 110033226_ipt_44_農田基地:3 ↔ 110033226_ipt_21_柵欄:1
- 貼合:12 [Mate]: 110033226_ipt_44_農田基地:3 ↔ 110033226_ipt_21_柵欄:13
- 貼合:13 [Mate]: 110033226_ipt_44_農田基地:3 ↔ 110033226_ipt_21_柵欄:13
- 貼合:14 [Mate]: 110033226_ipt_44_農田基地:3 ↔ 110033226_ipt_21_柵欄:13
- 貼合:15 [Mate]: 110033226_ipt_44_農田基地:3 ↔ 110033226_ipt_21_柵欄:16
- 貼合:16 [Mate]: 110033226_ipt_44_農田基地:3 ↔ 110033226_ipt_21_柵欄:16
- 貼合:17 [Mate]: 110033226_ipt_44_農田基地:3 ↔ 110033226_ipt_21_柵欄:16
- 貼合:18 [Mate]: 110033226_ipt_44_農田基地:3 ↔ 110033226_ipt_21_柵欄:14
- 貼合:19 [Mate]: 110033226_ipt_44_農田基地:3 ↔ 110033226_ipt_21_柵欄:14
- 貼合:20 [Mate]: 110033226_ipt_04_小河:3 ↔ 110033226_ipt_21_柵欄:14
- 貼合:21 [Mate]: 110033226_ipt_44_農田基地:3 ↔ 110033226_ipt_21_柵欄:15
- 貼合:22 [Mate]: 110033226_ipt_44_農田基地:3 ↔ 110033226_ipt_21_柵欄:15
- 貼合:23 [Mate]: 110033226_ipt_04_小河:15 ↔ 110033226_ipt_21_柵欄:15
- 貼合:24 [Mate]: 110033226_ipt_44_農田基地:3 ↔ 110033226_ipt_07_磚塊樺木(2x1):1
- 貼合:25 [Mate]: 110033226_ipt_44_農田基地:3 ↔ 110033226_ipt_07_磚塊樺木(2x1):1
- 貼合:26 [Mate]: 110033226_ipt_44_農田基地:3 ↔ 110033226_ipt_07_磚塊樺木(2x1):1
- 貼合:27 [Mate]: 110033226_ipt_44_農田基地:3 ↔ 110033226_ipt_07_磚塊樺木(2x1):3
- 貼合:28 [Mate]: 110033226_ipt_44_農田基地:3 ↔ 110033226_ipt_07_磚塊樺木(2x1):3
- 貼合:29 [Mate]: 110033226_ipt_44_農田基地:3 ↔ 110033226_ipt_07_磚塊樺木(2x1):3
- 貼合:30 [Mate]: 110033226_ipt_44_農田基地:3 ↔ 110033226_ipt_07_磚塊樺木(2x1):5
- 貼合:31 [Mate]: 110033226_ipt_44_農田基地:3 ↔ 110033226_ipt_07_磚塊樺木(2x1):5
- 貼合:32 [Mate]: 110033226_ipt_44_農田基地:3 ↔ 110033226_ipt_07_磚塊樺木(2x1):5
- 貼合:33 [Mate]: 110033226_ipt_44_農田基地:3 ↔ 110033226_ipt_07_磚塊樺木(2x1):2
- 貼合:34 [Mate]: 110033226_ipt_44_農田基地:3 ↔ 110033226_ipt_07_磚塊樺木(2x1):2
- 貼合:35 [Mate]: 110033226_ipt_44_農田基地:3 ↔ 110033226_ipt_07_磚塊樺木(2x1):2
- 貼合:36 [Mate]: 110033226_ipt_44_農田基地:3 ↔ 110033226_ipt_07_磚塊樺木(2x1):4
- 貼合:37 [Mate]: 110033226_ipt_44_農田基地:3 ↔ 110033226_ipt_07_磚塊樺木(2x1):4
- 貼合:38 [Mate]: 110033226_ipt_44_農田基地:3 ↔ 110033226_ipt_07_磚塊樺木(2x1):4
- 貼合:39 [Mate]: 110033226_ipt_44_農田基地:3 ↔ 110033226_ipt_13_草地二:1
- 貼合:40 [Mate]: 110033226_ipt_44_農田基地:3 ↔ 110033226_ipt_13_草地二:1
- 貼合:41 [Mate]: 110033226_ipt_44_農田基地:3 ↔ 110033226_ipt_13_草地二:1
- 貼合:42 [Mate]: 110033226_ipt_44_農田基地:3 ↔ 110033226_ipt_13_草地二:12
- 貼合:43 [Mate]: 110033226_ipt_44_農田基地:3 ↔ 110033226_ipt_13_草地二:12
- 貼合:44 [Mate]: 110033226_ipt_44_農田基地:3 ↔ 110033226_ipt_13_草地二:12
- 貼合:45 [Mate]: 110033226_ipt_44_農田基地:3 ↔ 110033226_ipt_13_草地二:11
- 貼合:46 [Mate]: 110033226_ipt_44_農田基地:3 ↔ 110033226_ipt_13_草地二:11
- 貼合:47 [Mate]: 110033226_ipt_44_農田基地:3 ↔ 110033226_ipt_13_草地二:11
- 貼合:48 [Mate]: 110033226_ipt_44_農田基地:3 ↔ 110033226_ipt_07_磚塊樺木(2x1):38
- 貼合:49 [Mate]: 110033226_ipt_44_農田基地:3 ↔ 110033226_ipt_07_磚塊樺木(2x1):38
- 貼合:50 [Mate]: 110033226_ipt_44_農田基地:3 ↔ 110033226_ipt_06_磚塊樺木(1x1):3
- 貼合:51 [Mate]: 110033226_ipt_07_磚塊樺木(2x1):38 ↔ 110033226_ipt_06_磚塊樺木(1x1):3
- 貼合:52 [Mate]: 110033226_ipt_07_磚塊樺木(2x1):38 ↔ 110033226_ipt_06_磚塊樺木(1x1):3
- 貼合:53 [Mate]: 110033226_ipt_06_磚塊樺木(1x1):11 ↔ 110033226_ipt_07_磚塊樺木(2x1):36
- 貼合:54 [Mate]: 110033226_ipt_06_磚塊樺木(1x1):11 ↔ 110033226_ipt_07_磚塊樺木(2x1):36
- 貼合:55 [Mate]: 110033226_ipt_07_磚塊樺木(2x1):46 ↔ 110033226_ipt_07_磚塊樺木(2x1):36
- 貼合:56 [Mate]: 110033226_ipt_07_磚塊樺木(2x1):46 ↔ 110033226_ipt_06_磚塊樺木(1x1):1
- 貼合:57 [Mate]: 110033226_ipt_07_磚塊樺木(2x1):36 ↔ 110033226_ipt_06_磚塊樺木(1x1):1